# Autodesk Inventor assembly: full
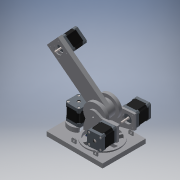
[picture p0: Inventor's stored thumbnail of the model, 180x180]
Saved by Autodesk Inventor 2019 (Build 230136000, 136)
## iProperties
Created: 2019-05-02
Part Number: full
Document SubType Name: Assembly
Designer: Nathan
Author: Nathan
## Documents named in this file (6)
- C:\Users\Nathan\workspace\fbd-brachium\cad\full.iam
- C:\Users\Nathan\workspace\fbd-brachium\cad\shoulder.ipt
- C:\Users\Nathan\workspace\fbd-brachium\cad\Nema17.ipt
- C:\Users\Nathan\workspace\fbd-brachium\cad\arm_proximal.ipt
- C:\Users\Nathan\workspace\fbd-brachium\cad\base.ipt
- C:\Users\Nathan\workspace\fbd-brachium\cad\parameters.xlsx
## Components (7 placed, 4 different names)
1. shoulder:1 — Insert:1, Insert:2, Insert:3, Insert:4, Insert:9, Insert:10
2. Nema17:1 — Insert:1, Insert:2
3. Nema17:2 — Insert:3, Insert:4
4. base:1 — Insert:9, Insert:13, Insert:14
5. arm_proximal:1 — Insert:10, Insert:11, Insert:12
6. Nema17:3 — Insert:11, Insert:12
7. Nema17:4 — Insert:13, Insert:14
## Relationships (10: Insert 10)
- Insert:1: shoulder:1 ↔ Nema17:1
- Insert:2: shoulder:1 ↔ Nema17:1
- Insert:3: shoulder:1 ↔ Nema17:2
- Insert:4: shoulder:1 ↔ Nema17:2
- Insert:9: shoulder:1 ↔ base:1
- Insert:10: shoulder:1 ↔ arm_proximal:1
- Insert:11: arm_proximal:1 ↔ Nema17:3
- Insert:12: arm_proximal:1 ↔ Nema17:3
- Insert:13: base:1 ↔ Nema17:4
- Insert:14: base:1 ↔ Nema17:4
## Named parameters: base_width = 165.1 mm, base_length = 127 mm, base_height = 12.7 mm, retention_poles_diameter = 6.35 mm, turntable_bed_depth = 6.35 mm, turntable_diameter = 101.6 mm, turntable_spur_thickness = 6.35 mm, turntable_thickness = 9.525 mm, spine_diameter = 38.1 mm, shoulder_height_offset = 25.4 mm, shoulder_width = 63.5 mm, shoulder_length = 50.8 mm, shoulder_wall_thickness = 6.35 mm, arm_proximal_gear_diameter = 63.5 mm, arm_proximal_gear_thickness = 9.525 mm, shoulder_motor_gear_diameter = 31.75 mm, arm_proximal_length = 177.8 mm, arm_proximal_width = 12.7 mm, waist_cutout_overlap = 6.35 mm, waist_motor_cutout_diameter = 50.8 mm, base_motor_standoff_thickness = 3.175 mm, base_motor_standoff_length = 63.5 mm, base_motor_standoff_height = 12.7 mm, base_motor_standoff_offset = 0 mm
